# Autodesk Inventor assembly: Unicycle
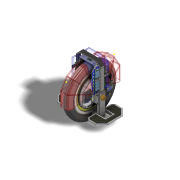
[picture p0: Inventor's stored thumbnail of the model, 180x180]
Saved by Autodesk Inventor 2020 (Build 240168000, 168)
## iProperties
Created: 2019-05-20
Part Number: Unicycle
Document SubType Name: Assembly
Designer: chitl
Author: chitl
## Documents named in this file (13)
- C:\Users\chitl\Desktop\OneWheel\Wheel Assembled\Unicycle.iam
- C:\Users\chitl\Desktop\OneWheel\Wheel Assembled\Wheel\Wheel.iam
- C:\Users\chitl\Desktop\OneWheel\Wheel Assembled\Pedal\Pedal.iam
- C:\Users\chitl\Desktop\OneWheel\Wheel Assembled\Chassis\Chassis.iam
- C:\Users\chitl\Desktop\OneWheel\Wheel Assembled\Battery Cover\Shell.ipt
- C:\Users\chitl\Documents\Inventor\Content Center Files\R2020\en-US\IFI (1)\IFI - I0.5625 - 12(1).ipt
- C:\Users\chitl\Desktop\OneWheel\Wheel Assembled\Chassis\Handle_Frame\Frame_Welded.iam
- C:\Users\chitl\Desktop\OneWheel\Wheel Assembled\Battery Cover\Battery Cover.ipt
- C:\Users\chitl\Desktop\OneWheel\Wheel Assembled\Sheet Metal Shell\Top.ipt
- C:\Users\chitl\Desktop\OneWheel\Wheel Assembled\Sheet Metal Shell\Shell_v2.ipt
- C:\Users\chitl\Desktop\OneWheel\Wheel Assembled\Handle\Handle Assembly.iam
- C:\Users\chitl\Documents\Inventor\Content Center Files\R2020\en-US\AS 1110\AS 1110 - M5 x 12.ipt
- C:\Users\chitl\Documents\Inventor\Content Center Files\R2020\en-US\AS 1110\AS 1110 - M2.5 x 10.ipt
## Components (22 placed, 12 different names)
1. Wheel:1 [sub-assembly] — Rotational:2, Rotational:3
2. Pedal:1 [sub-assembly] — Rotational:2, Flush:1, Rigid:1, Rigid:3, Mate:5, Mate:6
3. Pedal:2 [sub-assembly] — Rotational:3, Flush:1, Rigid:2, Mate:3, Mate:4, Mate:7
4. Chassis:1 [sub-assembly] — Rigid:3
5. Shell:1
6. Hex Flange Nut - Inch (IFI) I0.5625 - 12:1 — Rigid:1
7. Hex Flange Nut - Inch (IFI) I0.5625 - 12:2 — Rigid:2
8. Frame_Welded:1 [sub-assembly] — Mate:7, Insert:1, Insert:2, Insert:3, Insert:4
9. AS 1110 - Metric M5 x 12:1 — Mate:4
10. AS 1110 - Metric M5 x 12:2 — Mate:3
11. AS 1110 - Metric M5 x 12:3 — Mate:6
12. AS 1110 - Metric M5 x 12:4 — Mate:5
13. Battery Cover:1
14. Top:1
15. Top:2
16. Shell_v2:1
17. Shell_v2:2
18. Handle Assembly:1 [sub-assembly]
19. AS 1110 - Metric M2.5 x 10:1 — Insert:1
20. AS 1110 - Metric M2.5 x 10:2 — Insert:2
21. AS 1110 - Metric M2.5 x 10:3 — Insert:3
22. AS 1110 - Metric M2.5 x 10:4 — Insert:4
## Relationships (15: Mate 5, Insert 4, WeldJoint 3, RevoluteJoint 2, Flush 1)
- Rotational:2 [RevoluteJoint] (3.175 mm): Wheel:1 ↔ Pedal:1
- Rotational:3 [RevoluteJoint] (-3.175 mm): Wheel:1 ↔ Pedal:2
- Flush:1: Pedal:1 ↔ Pedal:2
- Rigid:1 [WeldJoint]: Pedal:1 ↔ Hex Flange Nut - Inch (IFI) I0.5625 - 12:1
- Rigid:2 [WeldJoint]: Pedal:2 ↔ Hex Flange Nut - Inch (IFI) I0.5625 - 12:2
- Rigid:3 [WeldJoint]: Pedal:1 ↔ Chassis:1
- Mate:3: Pedal:2 ↔ AS 1110 - Metric M5 x 12:2
- Mate:4: Pedal:2 ↔ AS 1110 - Metric M5 x 12:1
- Mate:5: Pedal:1 ↔ AS 1110 - Metric M5 x 12:4
- Mate:6: Pedal:1 ↔ AS 1110 - Metric M5 x 12:3
- Mate:7: Pedal:2 ↔ Frame_Welded:1
- Insert:1: Frame_Welded:1 ↔ AS 1110 - Metric M2.5 x 10:1
- Insert:2: Frame_Welded:1 ↔ AS 1110 - Metric M2.5 x 10:2
- Insert:3: Frame_Welded:1 ↔ AS 1110 - Metric M2.5 x 10:3
- Insert:4: Frame_Welded:1 ↔ AS 1110 - Metric M2.5 x 10:4
## Named parameters: sa_0 = 222411
note: some values were not read from the file. Shown as the stored number, unit unknown: "sa_0".
